# Autodesk Inventor assembly: Radio Power Module (REV-11-1856)
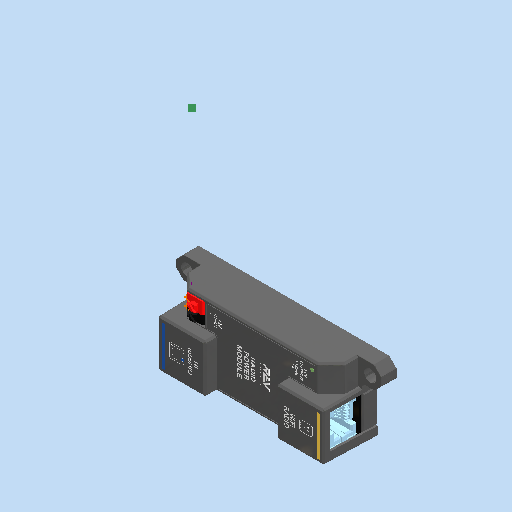
[picture p0: Inventor's stored thumbnail of the model, 512x512]
Saved by Autodesk Inventor 2023 (Build 270158000, 158)
## iProperties
Created: 2023-04-25
Part Number: Radio Power Module (REV-11-1856)
Document SubType Name: Assembly
Designer: jackc
Sending System: Onshape
FRU: Parasolid 34.1.198
FORMAT: text
GUISE: transmit
KEY: BTGapi::writeModels_.xmt
FILE: BTGapi::writeModels_.xmt
DATE: 2023-04-21T16:19:12 (UTC)
Author: jackc
## Documents named in this file (110)
- J:\My Drive\1939\2_Design\2023-2024\Parts\Electronics\Power Delivery\Radio Power Module (REV-11-1856).iam
- J:\My Drive\1939\2_Design\2023-2024\Parts\Electronics\RPM Parts\REV-11-1856.ipt
- J:\My Drive\1939\2_Design\2023-2024\Parts\Electronics\RPM Parts\REV-11-1856_1.ipt
- J:\My Drive\1939\2_Design\2023-2024\Parts\Electronics\RPM Parts\REV-11-1856_2.ipt
- J:\My Drive\1939\2_Design\2023-2024\Parts\Electronics\RPM Parts\REV-11-1856_3.ipt
- J:\My Drive\1939\2_Design\2023-2024\Parts\Electronics\RPM Parts\REV-11-1856_4.ipt
- J:\My Drive\1939\2_Design\2023-2024\Parts\Electronics\RPM Parts\REV-11-1856_5.ipt
- J:\My Drive\1939\2_Design\2023-2024\Parts\Electronics\RPM Parts\REV-11-1856_6.ipt
- J:\My Drive\1939\2_Design\2023-2024\Parts\Electronics\RPM Parts\REV-11-1856_7.ipt
- J:\My Drive\1939\2_Design\2023-2024\Parts\Electronics\RPM Parts\REV-11-1856_8.ipt
- J:\My Drive\1939\2_Design\2023-2024\Parts\Electronics\RPM Parts\REV-11-1856_9.ipt
- J:\My Drive\1939\2_Design\2023-2024\Parts\Electronics\RPM Parts\REV-11-1856_10.ipt
- J:\My Drive\1939\2_Design\2023-2024\Parts\Electronics\RPM Parts\REV-11-1856_11.ipt
- J:\My Drive\1939\2_Design\2023-2024\Parts\Electronics\RPM Parts\REV-11-1856_12.ipt
- J:\My Drive\1939\2_Design\2023-2024\Parts\Electronics\RPM Parts\REV-11-1856_13.ipt
- J:\My Drive\1939\2_Design\2023-2024\Parts\Electronics\RPM Parts\REV-11-1856_14.ipt
- J:\My Drive\1939\2_Design\2023-2024\Parts\Electronics\RPM Parts\REV-11-1856_15.ipt
- J:\My Drive\1939\2_Design\2023-2024\Parts\Electronics\RPM Parts\REV-11-1856_16.ipt
- J:\My Drive\1939\2_Design\2023-2024\Parts\Electronics\RPM Parts\REV-11-1856_17.ipt
- J:\My Drive\1939\2_Design\2023-2024\Parts\Electronics\RPM Parts\REV-11-1856_18.ipt
- J:\My Drive\1939\2_Design\2023-2024\Parts\Electronics\RPM Parts\REV-11-1856_19.ipt
- J:\My Drive\1939\2_Design\2023-2024\Parts\Electronics\RPM Parts\REV-11-1856_20.ipt
- J:\My Drive\1939\2_Design\2023-2024\Parts\Electronics\RPM Parts\REV-11-1856_21.ipt
- J:\My Drive\1939\2_Design\2023-2024\Parts\Electronics\RPM Parts\REV-11-1856_22.ipt
- J:\My Drive\1939\2_Design\2023-2024\Parts\Electronics\RPM Parts\REV-11-1856_23.ipt
- J:\My Drive\1939\2_Design\2023-2024\Parts\Electronics\RPM Parts\REV-11-1856_24.ipt
- J:\My Drive\1939\2_Design\2023-2024\Parts\Electronics\RPM Parts\REV-11-1856_25.ipt
- J:\My Drive\1939\2_Design\2023-2024\Parts\Electronics\RPM Parts\REV-11-1856_26.ipt
- J:\My Drive\1939\2_Design\2023-2024\Parts\Electronics\RPM Parts\REV-11-1856_27.ipt
- J:\My Drive\1939\2_Design\2023-2024\Parts\Electronics\RPM Parts\REV-11-1856_28.ipt
- J:\My Drive\1939\2_Design\2023-2024\Parts\Electronics\RPM Parts\REV-11-1856_29.ipt
- J:\My Drive\1939\2_Design\2023-2024\Parts\Electronics\RPM Parts\REV-11-1856_30.ipt
- J:\My Drive\1939\2_Design\2023-2024\Parts\Electronics\RPM Parts\REV-11-1856_31.ipt
- J:\My Drive\1939\2_Design\2023-2024\Parts\Electronics\RPM Parts\REV-11-1856_32.ipt
- J:\My Drive\1939\2_Design\2023-2024\Parts\Electronics\RPM Parts\REV-11-1856_33.ipt
- J:\My Drive\1939\2_Design\2023-2024\Parts\Electronics\RPM Parts\REV-11-1856_34.ipt
- J:\My Drive\1939\2_Design\2023-2024\Parts\Electronics\RPM Parts\REV-11-1856_35.ipt
- J:\My Drive\1939\2_Design\2023-2024\Parts\Electronics\RPM Parts\REV-11-1856_36.ipt
- J:\My Drive\1939\2_Design\2023-2024\Parts\Electronics\RPM Parts\REV-11-1856_37.ipt
- J:\My Drive\1939\2_Design\2023-2024\Parts\Electronics\RPM Parts\REV-11-1856_38.ipt
- J:\My Drive\1939\2_Design\2023-2024\Parts\Electronics\RPM Parts\REV-11-1856_39.ipt
- J:\My Drive\1939\2_Design\2023-2024\Parts\Electronics\RPM Parts\REV-11-1856_40.ipt
- J:\My Drive\1939\2_Design\2023-2024\Parts\Electronics\RPM Parts\REV-11-1856_41.ipt
- J:\My Drive\1939\2_Design\2023-2024\Parts\Electronics\RPM Parts\REV-11-1856_42.ipt
- J:\My Drive\1939\2_Design\2023-2024\Parts\Electronics\RPM Parts\REV-11-1856_43.ipt
- J:\My Drive\1939\2_Design\2023-2024\Parts\Electronics\RPM Parts\REV-11-1856_44.ipt
- J:\My Drive\1939\2_Design\2023-2024\Parts\Electronics\RPM Parts\REV-11-1856_45.ipt
- J:\My Drive\1939\2_Design\2023-2024\Parts\Electronics\RPM Parts\REV-11-1856_46.ipt
- J:\My Drive\1939\2_Design\2023-2024\Parts\Electronics\RPM Parts\REV-11-1856_48.ipt
- J:\My Drive\1939\2_Design\2023-2024\Parts\Electronics\RPM Parts\REV-11-1856_49.ipt
- J:\My Drive\1939\2_Design\2023-2024\Parts\Electronics\RPM Parts\REV-11-1856_50.ipt
- J:\My Drive\1939\2_Design\2023-2024\Parts\Electronics\RPM Parts\REV-11-1856_51.ipt
- J:\My Drive\1939\2_Design\2023-2024\Parts\Electronics\RPM Parts\REV-11-1856_52.ipt
- J:\My Drive\1939\2_Design\2023-2024\Parts\Electronics\RPM Parts\REV-11-1856_53.ipt
- J:\My Drive\1939\2_Design\2023-2024\Parts\Electronics\RPM Parts\REV-11-1856_54.ipt
- J:\My Drive\1939\2_Design\2023-2024\Parts\Electronics\RPM Parts\REV-11-1856_55.ipt
- J:\My Drive\1939\2_Design\2023-2024\Parts\Electronics\RPM Parts\REV-11-1856_56.ipt
- J:\My Drive\1939\2_Design\2023-2024\Parts\Electronics\RPM Parts\REV-11-1856_57.ipt
- J:\My Drive\1939\2_Design\2023-2024\Parts\Electronics\RPM Parts\REV-11-1856_58.ipt
- J:\My Drive\1939\2_Design\2023-2024\Parts\Electronics\RPM Parts\REV-11-1856_59.ipt
- J:\My Drive\1939\2_Design\2023-2024\Parts\Electronics\RPM Parts\REV-11-1856_60.ipt
- J:\My Drive\1939\2_Design\2023-2024\Parts\Electronics\RPM Parts\REV-11-1856_61.ipt
- J:\My Drive\1939\2_Design\2023-2024\Parts\Electronics\RPM Parts\REV-11-1856_62.ipt
- J:\My Drive\1939\2_Design\2023-2024\Parts\Electronics\RPM Parts\REV-11-1856_63.ipt
- J:\My Drive\1939\2_Design\2023-2024\Parts\Electronics\RPM Parts\REV-11-1856_64.ipt
- J:\My Drive\1939\2_Design\2023-2024\Parts\Electronics\RPM Parts\REV-11-1856_65.ipt
- J:\My Drive\1939\2_Design\2023-2024\Parts\Electronics\RPM Parts\REV-11-1856_66.ipt
- J:\My Drive\1939\2_Design\2023-2024\Parts\Electronics\RPM Parts\REV-11-1856_67.ipt
- J:\My Drive\1939\2_Design\2023-2024\Parts\Electronics\RPM Parts\REV-11-1856_68.ipt
- J:\My Drive\1939\2_Design\2023-2024\Parts\Electronics\RPM Parts\REV-11-1856_69.ipt
- J:\My Drive\1939\2_Design\2023-2024\Parts\Electronics\RPM Parts\REV-11-1856_70.ipt
- J:\My Drive\1939\2_Design\2023-2024\Parts\Electronics\RPM Parts\REV-11-1856_71.ipt
- J:\My Drive\1939\2_Design\2023-2024\Parts\Electronics\RPM Parts\REV-11-1856_72.ipt
- J:\My Drive\1939\2_Design\2023-2024\Parts\Electronics\RPM Parts\REV-11-1856_73.ipt
- J:\My Drive\1939\2_Design\2023-2024\Parts\Electronics\RPM Parts\REV-11-1856_74.ipt
- J:\My Drive\1939\2_Design\2023-2024\Parts\Electronics\RPM Parts\REV-11-1856_75.ipt
- J:\My Drive\1939\2_Design\2023-2024\Parts\Electronics\RPM Parts\REV-11-1856_76.ipt
- J:\My Drive\1939\2_Design\2023-2024\Parts\Electronics\RPM Parts\REV-11-1856_77.ipt
- J:\My Drive\1939\2_Design\2023-2024\Parts\Electronics\RPM Parts\REV-11-1856_78.ipt
- J:\My Drive\1939\2_Design\2023-2024\Parts\Electronics\RPM Parts\REV-11-1856_79.ipt
- J:\My Drive\1939\2_Design\2023-2024\Parts\Electronics\RPM Parts\REV-11-1856_80.ipt
- J:\My Drive\1939\2_Design\2023-2024\Parts\Electronics\RPM Parts\REV-11-1856_81.ipt
- J:\My Drive\1939\2_Design\2023-2024\Parts\Electronics\RPM Parts\REV-11-1856_82.ipt
- J:\My Drive\1939\2_Design\2023-2024\Parts\Electronics\RPM Parts\REV-11-1856_83.ipt
- J:\My Drive\1939\2_Design\2023-2024\Parts\Electronics\RPM Parts\REV-11-1856_84.ipt
- J:\My Drive\1939\2_Design\2023-2024\Parts\Electronics\RPM Parts\REV-11-1856_85.ipt
- J:\My Drive\1939\2_Design\2023-2024\Parts\Electronics\RPM Parts\REV-11-1856_86.ipt
- J:\My Drive\1939\2_Design\2023-2024\Parts\Electronics\RPM Parts\REV-11-1856_87.ipt
- J:\My Drive\1939\2_Design\2023-2024\Parts\Electronics\RPM Parts\REV-11-1856_88.ipt
- J:\My Drive\1939\2_Design\2023-2024\Parts\Electronics\RPM Parts\REV-11-1856_89.ipt
- J:\My Drive\1939\2_Design\2023-2024\Parts\Electronics\RPM Parts\REV-11-1856_90.ipt
- J:\My Drive\1939\2_Design\2023-2024\Parts\Electronics\RPM Parts\REV-11-1856_91.ipt
- J:\My Drive\1939\2_Design\2023-2024\Parts\Electronics\RPM Parts\REV-11-1856_92.ipt
- J:\My Drive\1939\2_Design\2023-2024\Parts\Electronics\RPM Parts\REV-11-1856_93.ipt
- J:\My Drive\1939\2_Design\2023-2024\Parts\Electronics\RPM Parts\REV-11-1856_94.ipt
- J:\My Drive\1939\2_Design\2023-2024\Parts\Electronics\RPM Parts\REV-11-1856_96.ipt
- J:\My Drive\1939\2_Design\2023-2024\Parts\Electronics\RPM Parts\REV-11-1856_97.ipt
- J:\My Drive\1939\2_Design\2023-2024\Parts\Electronics\RPM Parts\REV-11-1856_98.ipt
- J:\My Drive\1939\2_Design\2023-2024\Parts\Electronics\RPM Parts\REV-11-1856_99.ipt
- J:\My Drive\1939\2_Design\2023-2024\Parts\Electronics\RPM Parts\REV-11-1856_100.ipt
- J:\My Drive\1939\2_Design\2023-2024\Parts\Electronics\RPM Parts\REV-11-1856_101.ipt
- J:\My Drive\1939\2_Design\2023-2024\Parts\Electronics\RPM Parts\REV-11-1856_102.ipt
- J:\My Drive\1939\2_Design\2023-2024\Parts\Electronics\RPM Parts\REV-11-1856_103.ipt
- J:\My Drive\1939\2_Design\2023-2024\Parts\Electronics\RPM Parts\REV-11-1856_104.ipt
- J:\My Drive\1939\2_Design\2023-2024\Parts\Electronics\RPM Parts\REV-11-1856_105.ipt
- J:\My Drive\1939\2_Design\2023-2024\Parts\Electronics\RPM Parts\REV-11-1856_106.ipt
- J:\My Drive\1939\2_Design\2023-2024\Parts\Electronics\RPM Parts\REV-11-1856_107.ipt
- J:\My Drive\1939\2_Design\2023-2024\Parts\Electronics\RPM Parts\REV-11-1856_108.ipt
- J:\My Drive\1939\2_Design\2023-2024\Parts\Electronics\PDH Parts\Positive_small.ipt
- J:\My Drive\1939\2_Design\2023-2024\Parts\Electronics\PDH Parts\Negative_small.ipt
## Components (109 placed, 109 different names)
1. REV-11-1856
2. REV-11-1856_1
3. REV-11-1856_2
4. REV-11-1856_3
5. REV-11-1856_4
6. REV-11-1856_5
7. REV-11-1856_6
8. REV-11-1856_7
9. REV-11-1856_8
10. REV-11-1856_9
11. REV-11-1856_10
12. REV-11-1856_11
13. REV-11-1856_12
14. REV-11-1856_13 — Flush:1
15. REV-11-1856_14
16. REV-11-1856_15
17. REV-11-1856_16
18. REV-11-1856_17
19. REV-11-1856_18
20. REV-11-1856_19
21. REV-11-1856_20
22. REV-11-1856_21
23. REV-11-1856_22
24. REV-11-1856_23
25. REV-11-1856_24
26. REV-11-1856_25
27. REV-11-1856_26
28. REV-11-1856_27
29. REV-11-1856_28
30. REV-11-1856_29
31. REV-11-1856_30
32. REV-11-1856_31
33. REV-11-1856_32
34. REV-11-1856_33
35. REV-11-1856_34
36. REV-11-1856_35
37. REV-11-1856_36
38. REV-11-1856_37 — Mate:1, Flush:2
39. REV-11-1856_38
40. REV-11-1856_39
41. REV-11-1856_40
42. REV-11-1856_41
43. REV-11-1856_42
44. REV-11-1856_43
45. REV-11-1856_44
46. REV-11-1856_45
47. REV-11-1856_46
48. REV-11-1856_48
49. REV-11-1856_49
50. REV-11-1856_50
51. REV-11-1856_51
52. REV-11-1856_52
53. REV-11-1856_53
54. REV-11-1856_54
55. REV-11-1856_55
56. REV-11-1856_56
57. REV-11-1856_57
58. REV-11-1856_58
59. REV-11-1856_59
60. REV-11-1856_60
61. REV-11-1856_61
62. REV-11-1856_62
63. REV-11-1856_63
64. REV-11-1856_64
65. REV-11-1856_65
66. REV-11-1856_66
67. REV-11-1856_67
68. REV-11-1856_68
69. REV-11-1856_69
70. REV-11-1856_70
71. REV-11-1856_71
72. REV-11-1856_72
73. REV-11-1856_73
74. REV-11-1856_74
75. REV-11-1856_75
76. REV-11-1856_76
77. REV-11-1856_77
78. REV-11-1856_78
79. REV-11-1856_79
80. REV-11-1856_80
81. REV-11-1856_81
82. REV-11-1856_82
83. REV-11-1856_83
84. REV-11-1856_84
85. REV-11-1856_85
86. REV-11-1856_86
87. REV-11-1856_87
88. REV-11-1856_88
89. REV-11-1856_89
90. REV-11-1856_90
91. REV-11-1856_91
92. REV-11-1856_92
93. REV-11-1856_93
94. REV-11-1856_94
95. REV-11-1856_96
96. REV-11-1856_97
97. REV-11-1856_98
98. REV-11-1856_99
99. REV-11-1856_100
100. REV-11-1856_101
101. REV-11-1856_102
102. REV-11-1856_103
103. REV-11-1856_104
104. REV-11-1856_105
105. REV-11-1856_106
106. REV-11-1856_107
107. REV-11-1856_108
108. Positive_small:1 — Mate:1, Flush:1, Flush:2, Flush:3, Flush:4, Mate:2
109. Negative_small:1 — Flush:3, Flush:4, Mate:2
## Relationships (6: Flush 4, Mate 2)
- Mate:1: REV-11-1856_37 ↔ Positive_small:1
- Flush:1 (1.0414 mm): REV-11-1856_13 ↔ Positive_small:1
- Flush:2: REV-11-1856_37 ↔ Positive_small:1
- Flush:3: Positive_small:1 ↔ Negative_small:1
- Flush:4: Positive_small:1 ↔ Negative_small:1
- Mate:2: Positive_small:1 ↔ Negative_small:1
